# Autodesk Inventor assembly: arm
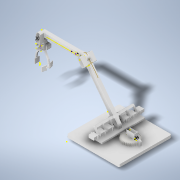
[picture p0: Inventor's stored thumbnail of the model, 180x180]
Saved by Autodesk Inventor 2021 (Build 250183000, 183)
## iProperties
Created: 2021-02-22
Part Number: arm
Document SubType Name: Assembly
Designer: josep
Author: josep
## Documents named in this file (14)
- C:\Users\josep\Documents\main_projects\Robot Arm\updated cad\arm.iam
- C:\Users\josep\Documents\main_projects\Robot Arm\updated cad\stationary gripper 7.ipt
- C:\Users\josep\Documents\main_projects\Robot Arm\updated cad\moving gripper 2.ipt
- C:\Users\josep\Documents\main_projects\Robot Arm\updated cad\wrist 3.ipt
- C:\Users\josep\Documents\main_projects\Robot Arm\updated cad\y arm 2.ipt
- C:\Users\josep\Documents\main_projects\Robot Arm\updated cad\bullet bill 1.ipt
- C:\Users\josep\Documents\main_projects\Robot Arm\updated cad\arm base holder 1.ipt
- C:\Users\josep\Documents\main_projects\Robot Arm\updated cad\servo holder 2.ipt
- C:\Users\josep\Documents\main_projects\Robot Arm\updated cad\wood part 1.ipt
- C:\Users\josep\Documents\main_projects\Robot Arm\updated cad\Spur Gears6.iam
- C:\Users\josep\Documents\main_projects\Robot Arm\updated cad\wood part 2.ipt
- C:\Users\josep\Documents\main_projects\Robot Arm\updated cad\x arm 2.ipt
- C:\Users\josep\Documents\main_projects\Robot Arm\updated cad\servo placeholder.ipt
- C:\Users\josep\Documents\main_projects\Robot Arm\updated cad\y arm connection.ipt
## Components (18 placed, 13 different names)
1. stationary gripper 7:1
2. moving gripper 2:1
3. wrist 3:1
4. y arm 2:1
5. bullet bill 1:1
6. arm base holder 1:1
7. Spur Gears:1 [sub-assembly]
8. servo holder 2:7
9. wood part 2:1
10. x arm 2:1
11. wood part 1:1
12. servo placeholder:1 — Flush:7, Flush:10
13. servo placeholder:2 — Flush:6, Flush:7, Flush:9, Flush:10
14. servo placeholder:3 — Flush:5, Flush:6, Flush:8, Flush:9
15. servo placeholder:4 — Flush:1, Flush:3, Flush:5, Flush:8
16. servo placeholder:5 — Flush:1, Flush:2, Flush:3, Flush:4
17. servo placeholder:6 — Flush:2, Flush:4
18. y arm connection:1
## Relationships (10: Flush 10)
- Flush:1: servo placeholder:4 ↔ servo placeholder:5
- Flush:2: servo placeholder:5 ↔ servo placeholder:6
- Flush:3: servo placeholder:4 ↔ servo placeholder:5
- Flush:4: servo placeholder:5 ↔ servo placeholder:6
- Flush:5: servo placeholder:3 ↔ servo placeholder:4
- Flush:6: servo placeholder:2 ↔ servo placeholder:3
- Flush:7: servo placeholder:1 ↔ servo placeholder:2
- Flush:8: servo placeholder:3 ↔ servo placeholder:4
- Flush:9: servo placeholder:2 ↔ servo placeholder:3
- Flush:10: servo placeholder:1 ↔ servo placeholder:2
